# Autodesk Inventor assembly: GP6-200v2
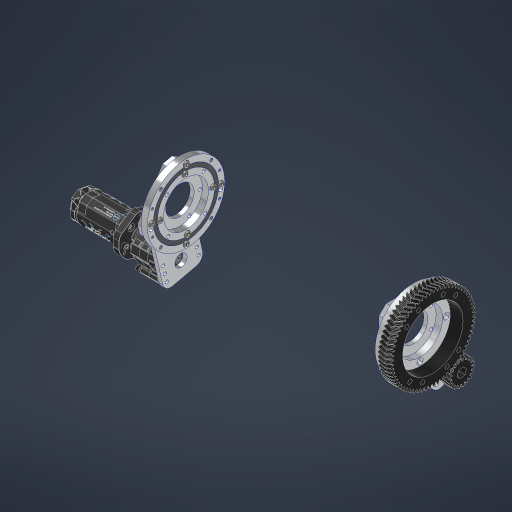
[picture p0: Inventor's stored thumbnail of the model, 512x512]
Saved by Autodesk Inventor 2023.4 (Build 274418000, 418)
## iProperties
Created: 2025-02-23
Part Number: GP6-200v2
Document SubType Name: Assembly
Designer: brand
Author: brand
## Documents named in this file (10)
- C:\Users\brand\OneDrive\Documents\GitHub\robotics 23\2025-ReefScape---CAD\Gripper\GP6\GP6-200v2.iam
- C:\Users\brand\OneDrive\Documents\GitHub\robotics 23\2025-ReefScape---CAD\Gripper\GP6\GP6-004.ipt
- C:\Users\brand\OneDrive\Documents\GitHub\robotics 23\2025-ReefScape---CAD\COMMON PARTS\4in Lazy Suzan.iam
- C:\Users\brand\OneDrive\Documents\GitHub\robotics 23\2025-ReefScape---CAD\COMMON PARTS\GEARS\Herringbone\2m 64t herringbone\2m 64t herringbone.ipt
- C:\Users\brand\OneDrive\Documents\GitHub\robotics 23\2025-ReefScape---CAD\COMMON PARTS\GEARBOXES\MAX Planetary\MAX Planetary Configurable 9-1 Kraken x44\MAX Planetary Configurable 9-1 Kraken x44.iam
- C:\Users\brand\OneDrive\Documents\GitHub\robotics 23\2025-ReefScape---CAD\COMMON PARTS\GEARS\Herringbone\2m 18t herringbone\2m 18t herringbone.ipt
- C:\Users\brand\OneDrive\Documents\GitHub\robotics 23\2025-ReefScape---CAD\COMMON PARTS\REV Robotics\hall effect switch assembly.iam
- C:\Users\brand\OneDrive\Documents\GitHub\robotics 23\2025-ReefScape---CAD\Gripper\GP7\GP7-006.ipt
- C:\Users\brand\OneDrive\Documents\GitHub\robotics 23\2025-ReefScape---CAD\Arm\AR-020.ipt
- C:\Users\brand\OneDrive\Documents\GitHub\robotics 23\2025-ReefScape---CAD\COMMON PARTS\Lazy Suzan\LS1-100.iam
## Components (9 placed, 9 different names)
1. GP6-004:1 — Mate:1, Insert:7, Insert:8, Insert:15, Insert:17, Insert:18, Insert:19
2. 4in Lazy Suzan:1 [sub-assembly] — Rotation:1, Insert:7, Insert:8, Insert:9, Insert:10
3. 2m 64t herringbone:1 — Flush:1, Insert:9, Insert:10
4. MAX Planetary Configurable 9-1 Kraken x44:1 [sub-assembly] — Insert:24
5. 2m 18t herringbone:1 — Mate:1, Flush:1, Rotation:1
6. hall effect switch assembly:1 [sub-assembly] — Insert:14, Insert:16, Insert:22, Insert:23
7. GP7-006:1 — Insert:14, Insert:15, Insert:16, Insert:17
8. AR-020:1 — Insert:18, Insert:19, Insert:22, Insert:23
9. LS1-100:2 [sub-assembly] — Insert:24
## Relationships (16: Insert 13, Mate 1, Flush 1, RelateRotation 1)
- Mate:1: GP6-004:1 ↔ 2m 18t herringbone:1
- Flush:1: 2m 64t herringbone:1 ↔ 2m 18t herringbone:1
- Rotation:1 [RelateRotation] (3.5556 ul): 4in Lazy Suzan:1 ↔ 2m 18t herringbone:1
- Insert:7: GP6-004:1 ↔ 4in Lazy Suzan:1
- Insert:8: GP6-004:1 ↔ 4in Lazy Suzan:1
- Insert:9: 4in Lazy Suzan:1 ↔ 2m 64t herringbone:1
- Insert:10: 4in Lazy Suzan:1 ↔ 2m 64t herringbone:1
- Insert:14: hall effect switch assembly:1 ↔ GP7-006:1
- Insert:15: GP6-004:1 ↔ GP7-006:1
- Insert:16: hall effect switch assembly:1 ↔ GP7-006:1
- Insert:17: GP6-004:1 ↔ GP7-006:1
- Insert:18: GP6-004:1 ↔ AR-020:1
- Insert:19: GP6-004:1 ↔ AR-020:1
- Insert:22: hall effect switch assembly:1 ↔ AR-020:1
- Insert:23: hall effect switch assembly:1 ↔ AR-020:1
- Insert:24: MAX Planetary Configurable 9-1 Kraken x44:1 ↔ LS1-100:2
